# Autodesk Inventor assembly: 2axisRotator
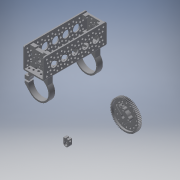
[picture p0: Inventor's stored thumbnail of the model, 180x180]
Saved by Autodesk Inventor 2018 (Build 220112000, 112)
## iProperties
Created: 2017-10-12
Part Number: 2axisRotator
Document SubType Name: Assembly
Designer: ball
Author: ball
## Documents named in this file (9)
- C:\FTC\2017 Robot\TestInventor\2axisRotator.iam
- C:\FTC\PTC Creo\Actobotics\535 parts\535130 assembly.ipt
- C:\FTC\PTC Creo\Actobotics\555 parts\555116.ipt
- C:\FTC\PTC Creo\Actobotics\625 parts\625102.ipt
- C:\FTC\PTC Creo\Actobotics\615 parts\615194.ipt
- C:\FTC\PTC Creo\Actobotics\545 parts\545619 assembly.ipt
- C:\FTC\PTC Creo\Actobotics\585 parts\585444.ipt
- C:\FTC\PTC Creo\Actobotics\545 parts\545360.ipt
- C:\FTC\PTC Creo\Actobotics\535 parts\535198.ipt
## Components (9 placed, 8 different names)
1. 585444:2 — Mate:3, Mate:4, Mate:5, Mate:6, Mate:7, Mate:8, Mate:9, Mate:10, Mate:11, Mate:12, Mate:13, Mate:14
2. 535130 assembly:2 — Mate:9, Mate:10, Mate:11
3. 555116:1 — Mate:6, Mate:7, Mate:8
4. 555116:2 — Mate:3, Mate:4, Mate:5
5. 625102:1
6. 615194:1 — Insert:8, Mate:1
7. 545619 assembly:2 — Insert:8, Mate:1
8. 545360:1 — Mate:12, Mate:13, Mate:14, Mate:15, Mate:16
9. 535198:1 — Mate:15, Mate:16
## Relationships (16: Mate 15, Insert 1)
- Insert:8: 615194:1 ↔ 545619 assembly:2
- Mate:1: 615194:1 ↔ 545619 assembly:2
- Mate:3: 585444:2 ↔ 555116:2
- Mate:4: 585444:2 ↔ 555116:2
- Mate:5: 585444:2 ↔ 555116:2
- Mate:6: 585444:2 ↔ 555116:1
- Mate:7: 585444:2 ↔ 555116:1
- Mate:8: 585444:2 ↔ 555116:1
- Mate:9: 585444:2 ↔ 535130 assembly:2
- Mate:10: 585444:2 ↔ 535130 assembly:2
- Mate:11: 585444:2 ↔ 535130 assembly:2
- Mate:12: 585444:2 ↔ 545360:1
- Mate:13: 585444:2 ↔ 545360:1
- Mate:14: 585444:2 ↔ 545360:1
- Mate:15: 545360:1 ↔ 535198:1
- Mate:16: 545360:1 ↔ 535198:1
